# Autodesk Inventor assembly: Assembly1
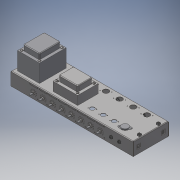
[picture p0: Inventor's stored thumbnail of the model, 180x180]
Saved by Autodesk Inventor 2016 (Build 200138000, 138)
## iProperties
Created: 2015-10-14
Part Number: Assembly1
Document SubType Name: Assembly
Designer: jeremyhale
Author: jeremyhale
## Documents named in this file (33)
- \\psf\Home\Documents\Poorhouse\git\p0001\chassis.iam
- chassis.iam
- \\psf\Home\Documents\Poorhouse\git\p0001\tube socket 8 pin.ipt
- \\psf\Home\Documents\Poorhouse\git\p0001\tube socket 9 pin.ipt
- \\psf\Home\Documents\Poorhouse\git\p0001\xmfr power.ipt
- \\psf\Home\Documents\Poorhouse\git\p0001\xmfr output.ipt
- \\psf\Home\Documents\Inventor\Content Center Files\R2016\en-US\AS 1474(1)\AS 1474 - M3(1).ipt
- \\psf\Home\Documents\Poorhouse\git\p0001\iec320_703W-00_04.ipt
- \\psf\Home\Documents\Inventor\Content Center Files\R2016\en-US\AS 1427(07)\AS 1427 - M3 x 10(6) II.ipt
- \\psf\Home\Documents\Poorhouse\git\p0001\Toggle Large A.ipt
- \\psf\Home\Documents\Poorhouse\git\p0001\AUDIO JACK 2.ipt
- \\psf\Home\Documents\Poorhouse\git\p0001\Bussman fuse holder HKP - 0,25'' X 1,25''.ipt
- \\psf\Home\Documents\Poorhouse\git\p0001\cage nut m6.iam
- \\psf\Home\Documents\Poorhouse\git\p0001\PEC11R-4220F-S0024.ipt
- \\psf\Home\Documents\Inventor\Content Center Files\R2016\en-US\UNI 5590  A\UNI 5590 - A M7.ipt
- \\psf\Home\Documents\Inventor\Content Center Files\R2016\en-US\BS 4320(2)\BS 4320 - M7 (Form B).ipt
- \\psf\Home\Documents\Poorhouse\git\p0001\rotary control.iam
- \\psf\Home\Documents\Poorhouse\git\p0001\Standoff 7mm M2 Wurth 9774070243R.ipt
- \\psf\Home\Documents\Poorhouse\git\p0001\chassis\Design Accelerator\Bolted Connection2.iam
- \\psf\Home\Documents\Poorhouse\git\p0001\chassis\Design Accelerator\Bolted Connection3.iam
- \\psf\Home\Documents\Poorhouse\git\p0001\chassis\Design Accelerator\Bolted Connection4.iam
- \\psf\Home\Documents\Poorhouse\git\p0001\chassis\Design Accelerator\Bolted Connection5.iam
- \\psf\Home\Documents\Poorhouse\git\p0001\chassis\Design Accelerator\Bolted Connection8.iam
- \\psf\Home\Documents\Poorhouse\git\p0001\chassis-weld.iam
- \\psf\Home\Documents\Poorhouse\git\p0001\octal assembly.ipt
- \\psf\Home\Documents\Poorhouse\git\p0001\chassis\Design Accelerator\Bolted Connection6.iam
- \\psf\Home\Documents\Poorhouse\git\p0001\el34 assembly_r1.ipt
- \\psf\Home\Documents\Poorhouse\git\p0001\chassis\Design Accelerator\Bolted Connection7.iam
- \\psf\Home\Documents\Poorhouse\git\p0001\chassis\Design Accelerator\Bolted Connection9.iam
- \\psf\Home\Documents\Poorhouse\git\p0001\Noval socket.ipt
- \\psf\Home\Documents\Poorhouse\git\p0001\12ax7_complete.ipt
- \\psf\Home\Documents\Poorhouse\git\p0001\chassis\Design Accelerator\Bolted Connection10.iam
- \\psf\Home\Documents\Poorhouse\git\p0001\chassis\Design Accelerator\Bolted Connection14.iam
## Components (204 placed, 25 different names)
1. xmfr power:1 — Mate:55, Mate:77, Flush:7, Flush:8, Mate:108, Mate:109
2. xmfr output:1 — Mate:76, Mate:77, Flush:6, Mate:110, Mate:111
3. Bussman fuse holder HKP - 0,25'' X 1,25'':1
4. PowerSwitch
5. chassis-weld:1 [sub-assembly] — Angle:1, Rotational:29, Rotational:30, Insert:43, Angle:2, Rigid:32, Insert:44, Angle:3, Insert:45, Angle:4, Mate:55, Mate:76, Flush:6, Flush:7, Flush:8, Mate:112, Mate:113, Mate:114, Mate:115, Mate:116, Mate:117, Mate:118, Rigid:36, Mate:119, Mate:120
6. big preamp tube socket — Insert:44, Angle:3, Mate:51, Mate:52
7. Bolted Connection:113 [sub-assembly] — Mate:108, Mate:109
8. Bolted Connection:117 [sub-assembly] — Mate:110, Mate:111
9. iec320_703W-00_04:1 — Mate:6, Mate:7
10. AS 1427 Z - Metric M3 x 10:2 — Mate:6, Mate:10
11. AS 1427 Z - Metric M3 x 10:1 — Mate:7, Mate:12
12. AS 1474 - Metric M3:5 — Mate:10
13. AS 1474 - Metric M3:6 — Mate:12
14. Input Jack
15. AUDIO JACK 2:5
16. Bolted Connection:4 [sub-assembly] — Mate:38
17. Bolted Connection:3 [sub-assembly] — Mate:30
18. Bolted Connection:2 [sub-assembly] — Mate:32
19. Bolted Connection:1 [sub-assembly] — Mate:34
20. Standoff 7mm M2 Wurth 9774070243R:4 — Insert:42, Mate:38
21. Standoff 7mm M2 Wurth 9774070243R:3 — Insert:41, Mate:32
22. Standoff 7mm M2 Wurth 9774070243R:2 — Insert:40, Mate:30
23. Standoff 7mm M2 Wurth 9774070243R:1 — Insert:39, Mate:34
24. rotary control:1 [sub-assembly] — Insert:39, Insert:40, Insert:41, Insert:42, Angle:1, Cylindrical:1, Mate:39, Mate:40
25. BS 4320 Form AB M7 (Form B):1 — Mate:15, Mate:18
26. UNI 5590 A A M7:1 — Mate:17, Mate:18
27. PEC11R-4220F-S0024:1 — Mate:15, Mate:17, Cylindrical:1
28. Bolted Connection:37 [sub-assembly]
29. Bolted Connection:38 [sub-assembly]
30. Bolted Connection:39 [sub-assembly]
31. Bolted Connection:40 [sub-assembly]
32. Standoff 7mm M2 Wurth 9774070243R:5
33. Standoff 7mm M2 Wurth 9774070243R:6
34. Standoff 7mm M2 Wurth 9774070243R:7
35. Standoff 7mm M2 Wurth 9774070243R:8
36. rotary control:2 [sub-assembly]
37. BS 4320 Form AB M7 (Form B):2
38. UNI 5590 A A M7:2
39. PEC11R-4220F-S0024:2
40. Bolted Connection:45 [sub-assembly]
41. Bolted Connection:46 [sub-assembly]
42. Bolted Connection:47 [sub-assembly]
43. Bolted Connection:48 [sub-assembly]
44. Standoff 7mm M2 Wurth 9774070243R:9
45. Standoff 7mm M2 Wurth 9774070243R:10
46. Standoff 7mm M2 Wurth 9774070243R:11
47. Standoff 7mm M2 Wurth 9774070243R:12
48. rotary control:3 [sub-assembly]
49. BS 4320 Form AB M7 (Form B):3
50. UNI 5590 A A M7:3
51. PEC11R-4220F-S0024:3
52. Bolted Connection:53 [sub-assembly]
53. Bolted Connection:54 [sub-assembly]
54. Bolted Connection:55 [sub-assembly]
55. Bolted Connection:56 [sub-assembly]
56. Standoff 7mm M2 Wurth 9774070243R:13
57. Standoff 7mm M2 Wurth 9774070243R:14
58. Standoff 7mm M2 Wurth 9774070243R:15
59. Standoff 7mm M2 Wurth 9774070243R:16
60. rotary control:4 [sub-assembly]
61. BS 4320 Form AB M7 (Form B):4
62. UNI 5590 A A M7:4
63. PEC11R-4220F-S0024:4
64. Bolted Connection:61 [sub-assembly]
65. Bolted Connection:62 [sub-assembly]
66. Bolted Connection:63 [sub-assembly]
67. Bolted Connection:64 [sub-assembly]
68. Standoff 7mm M2 Wurth 9774070243R:17
69. Standoff 7mm M2 Wurth 9774070243R:18
70. Standoff 7mm M2 Wurth 9774070243R:19
71. Standoff 7mm M2 Wurth 9774070243R:20
72. rotary control:5 [sub-assembly]
73. BS 4320 Form AB M7 (Form B):5
74. UNI 5590 A A M7:5
75. PEC11R-4220F-S0024:5
76. Bolted Connection:69 [sub-assembly]
77. Bolted Connection:70 [sub-assembly]
78. Bolted Connection:71 [sub-assembly]
79. Bolted Connection:72 [sub-assembly]
80. Standoff 7mm M2 Wurth 9774070243R:21
81. Standoff 7mm M2 Wurth 9774070243R:22
82. Standoff 7mm M2 Wurth 9774070243R:23
83. Standoff 7mm M2 Wurth 9774070243R:24
84. rotary control:6 [sub-assembly]
85. BS 4320 Form AB M7 (Form B):6
86. UNI 5590 A A M7:6
87. PEC11R-4220F-S0024:6
88. Bolted Connection:77 [sub-assembly]
89. Bolted Connection:78 [sub-assembly]
90. Bolted Connection:79 [sub-assembly]
91. Bolted Connection:80 [sub-assembly]
92. Standoff 7mm M2 Wurth 9774070243R:25
93. Standoff 7mm M2 Wurth 9774070243R:26
94. Standoff 7mm M2 Wurth 9774070243R:27
95. Standoff 7mm M2 Wurth 9774070243R:28
96. rotary control:7 [sub-assembly]
97. BS 4320 Form AB M7 (Form B):7
98. UNI 5590 A A M7:7
99. PEC11R-4220F-S0024:7
100. Bolted Connection:85 [sub-assembly]
101. Bolted Connection:86 [sub-assembly]
102. Bolted Connection:87 [sub-assembly]
103. Bolted Connection:88 [sub-assembly]
104. Standoff 7mm M2 Wurth 9774070243R:29
105. Standoff 7mm M2 Wurth 9774070243R:30
106. Standoff 7mm M2 Wurth 9774070243R:31
107. Standoff 7mm M2 Wurth 9774070243R:32
108. rotary control:8 [sub-assembly]
109. BS 4320 Form AB M7 (Form B):8
110. UNI 5590 A A M7:8
111. PEC11R-4220F-S0024:8
112. AUDIO JACK 2:6 — Rotational:29
113. AUDIO JACK 2:7
114. AUDIO JACK 2:8
115. jack speaker — Rotational:30
116. AUDIO JACK 2:9
117. AUDIO JACK 2:10
118. tube socket 8 pin:1 — Insert:43, Angle:2, Mate:53, Mate:54
119. octal assembly:1 — Rigid:32, Rigid:33
120. el34 assembly_r1:1 — Rigid:33
121. tube socket 8 pin:8
122. octal assembly:2
123. el34 assembly_r1:2
124. tube socket 8 pin:9
125. octal assembly:3
126. el34 assembly_r1:3
127. tube socket 8 pin:10
128. octal assembly:4
129. el34 assembly_r1:4
130. tube socket 8 pin:11
131. octal assembly:5
132. el34 assembly_r1:5
133. tube socket 8 pin:12
134. octal assembly:6
135. el34 assembly_r1:6
136. Bolted Connection:105 [sub-assembly] — Mate:51, Mate:52
137. Bolted Connection:106 [sub-assembly]
138. tube socket 9 pin:1 — Insert:45, Angle:4, Mate:49, Mate:50
139. Noval socket:1 — Rigid:35, Rigid:36
140. 12ax7_complete:1 — Rigid:35
141. tube socket 9 pin:2
142. Noval socket:2
143. 12ax7_complete:2
144. tube socket 9 pin:3
145. Noval socket:3
146. 12ax7_complete:3
147. cage nut m6:5 [sub-assembly] — Mate:112, Mate:113, Mate:114
148. cage nut m6:9 [sub-assembly]
149. cage nut m6:7 [sub-assembly] — Mate:115, Mate:116, Mate:117
150. cage nut m6:10 [sub-assembly]
151. cage nut m6:1 [sub-assembly] — Mate:118, Mate:119, Mate:120
152. cage nut m6:11 [sub-assembly]
153. cage nut m6:12 [sub-assembly]
154. cage nut m6:13 [sub-assembly]
155. Bolted Connection:33 [sub-assembly] — Mate:39, Mate:40
156. Bolted Connection:34 [sub-assembly]
157. Bolted Connection:35 [sub-assembly]
158. Bolted Connection:36 [sub-assembly]
159. Bolted Connection:41 [sub-assembly]
160. Bolted Connection:42 [sub-assembly]
161. Bolted Connection:43 [sub-assembly]
162. Bolted Connection:44 [sub-assembly]
163. Bolted Connection:49 [sub-assembly]
164. Bolted Connection:50 [sub-assembly]
165. Bolted Connection:51 [sub-assembly]
166. Bolted Connection:52 [sub-assembly]
167. Bolted Connection:57 [sub-assembly]
168. Bolted Connection:58 [sub-assembly]
169. Bolted Connection:59 [sub-assembly]
170. Bolted Connection:60 [sub-assembly]
171. Bolted Connection:65 [sub-assembly]
172. Bolted Connection:66 [sub-assembly]
173. Bolted Connection:67 [sub-assembly]
174. Bolted Connection:68 [sub-assembly]
175. Bolted Connection:73 [sub-assembly]
176. Bolted Connection:74 [sub-assembly]
177. Bolted Connection:75 [sub-assembly]
178. Bolted Connection:76 [sub-assembly]
179. Bolted Connection:81 [sub-assembly]
180. Bolted Connection:82 [sub-assembly]
181. Bolted Connection:83 [sub-assembly]
182. Bolted Connection:84 [sub-assembly]
183. Bolted Connection:89 [sub-assembly]
184. Bolted Connection:90 [sub-assembly]
185. Bolted Connection:91 [sub-assembly]
186. Bolted Connection:92 [sub-assembly]
187. Bolted Connection:93 [sub-assembly] — Mate:53, Mate:54
188. Bolted Connection:94 [sub-assembly]
189. Bolted Connection:95 [sub-assembly]
190. Bolted Connection:96 [sub-assembly]
191. Bolted Connection:97 [sub-assembly]
192. Bolted Connection:98 [sub-assembly]
193. Bolted Connection:99 [sub-assembly]
194. Bolted Connection:100 [sub-assembly]
195. Bolted Connection:101 [sub-assembly]
196. Bolted Connection:102 [sub-assembly]
197. Bolted Connection:103 [sub-assembly]
198. Bolted Connection:104 [sub-assembly]
199. Bolted Connection:107 [sub-assembly] — Mate:49, Mate:50
200. Bolted Connection:108 [sub-assembly]
201. Bolted Connection:109 [sub-assembly]
202. Bolted Connection:110 [sub-assembly]
203. Bolted Connection:111 [sub-assembly]
204. Bolted Connection:112 [sub-assembly]
## Component patterns: jacks input (2 elements), controls (8 elements), jacks fx (3 elements), jacks speaker (3 elements), big tubes (6 elements), big preamp tube screws (2 elements), small preamp tubes (3 elements), (2 elements, first: cage nut m6:5), (2 elements, first: cage nut m6:7), (4 elements, first: cage nut m6:1), (4 elements, first: Bolted Connection:33), Component Pattern 21:2 (4 elements), Component Pattern 21:3 (4 elements), Component Pattern 21:4 (4 elements), Component Pattern 21:5 (4 elements), Component Pattern 21:6 (4 elements), Component Pattern 21:7 (4 elements), Component Pattern 21:8 (4 elements), big tube socket screws (2 elements), big tube socket screws:2 (2 elements), big tube socket screws:3 (2 elements), big tube socket screws:4 (2 elements), big tube socket screws:5 (2 elements), big tube socket screws:6 (2 elements), small tube screws (2 elements), small tube screws:2 (2 elements), small tube screws:3 (2 elements)
## Relationships (74: Mate 44, Insert 7, RevoluteJoint 6, WeldJoint 6, Flush 6, Angle 4, CylindricalJoint 1)
- [RevoluteJoint]: chassis-weld:1 ↔ iec320_703W-00_04:1
- [RevoluteJoint]: chassis-weld:1 ↔ iec320_703W-00_04:1
- Mate:6: iec320_703W-00_04:1 ↔ AS 1427 Z - Metric M3 x 10:2
- Mate:7: iec320_703W-00_04:1 ↔ AS 1427 Z - Metric M3 x 10:1
- Mate:10: AS 1427 Z - Metric M3 x 10:2 ↔ AS 1474 - Metric M3:5
- [Mate]: chassis-weld:1 ↔ AS 1474 - Metric M3:5
- Mate:12: AS 1427 Z - Metric M3 x 10:1 ↔ AS 1474 - Metric M3:6
- [Mate]: chassis-weld:1 ↔ AS 1474 - Metric M3:6
- [WeldJoint]: Bussman fuse holder HKP - 0,25'' X 1,25'':1 ↔ chassis-weld:1
- [WeldJoint]: PowerSwitch ↔ chassis-weld:1
- [Flush]: chassis-weld:1
- [Flush]: chassis-weld:1
- [Flush]: chassis-weld:1
- Mate:15: BS 4320 Form AB M7 (Form B):1 ↔ PEC11R-4220F-S0024:1
- [Mate]: chassis-weld:1 ↔ BS 4320 Form AB M7 (Form B):1
- Mate:17: UNI 5590 A A M7:1 ↔ PEC11R-4220F-S0024:1
- Mate:18: BS 4320 Form AB M7 (Form B):1 ↔ UNI 5590 A A M7:1
- Insert:39: Standoff 7mm M2 Wurth 9774070243R:1 ↔ rotary control:1
- Insert:40: Standoff 7mm M2 Wurth 9774070243R:2 ↔ rotary control:1
- Insert:41: Standoff 7mm M2 Wurth 9774070243R:3 ↔ rotary control:1
- Insert:42: Standoff 7mm M2 Wurth 9774070243R:4 ↔ rotary control:1
- [Mate]: chassis-weld:1 ↔ Standoff 7mm M2 Wurth 9774070243R:1
- [Mate]: chassis-weld:1 ↔ Standoff 7mm M2 Wurth 9774070243R:4
- Angle:1 (0 deg): chassis-weld:1 ↔ rotary control:1
- Cylindrical:1: rotary control:1 ↔ PEC11R-4220F-S0024:1
- [Mate]: chassis-weld:1 ↔ Bolted Connection:3
- Mate:30: Bolted Connection:3 ↔ Standoff 7mm M2 Wurth 9774070243R:2
- [Mate]: chassis-weld:1 ↔ Bolted Connection:2
- Mate:32: Bolted Connection:2 ↔ Standoff 7mm M2 Wurth 9774070243R:3
- [Mate]: chassis-weld:1 ↔ Bolted Connection:1
- Mate:34: Bolted Connection:1 ↔ Standoff 7mm M2 Wurth 9774070243R:1
- [RevoluteJoint]: chassis-weld:1 ↔ Input Jack
- [RevoluteJoint]: chassis-weld:1 ↔ PEC11R-4220F-S0024:1
- [Mate]: chassis-weld:1 ↔ Bolted Connection:4
- Mate:38: Bolted Connection:4 ↔ Standoff 7mm M2 Wurth 9774070243R:4
- Mate:39: rotary control:1 ↔ Bolted Connection:33
- Mate:40: rotary control:1 ↔ Bolted Connection:33
- Rotational:29 [RevoluteJoint]: chassis-weld:1 ↔ AUDIO JACK 2:6
- Rotational:30 [RevoluteJoint]: chassis-weld:1 ↔ jack speaker
- Insert:43: chassis-weld:1 ↔ tube socket 8 pin:1
- Angle:2 (120 deg): chassis-weld:1 ↔ tube socket 8 pin:1
- Rigid:32 [WeldJoint]: chassis-weld:1 ↔ octal assembly:1
- Rigid:33 [WeldJoint]: octal assembly:1 ↔ el34 assembly_r1:1
- Insert:44: chassis-weld:1 ↔ big preamp tube socket
- Angle:3 (30 deg): chassis-weld:1 ↔ big preamp tube socket
- Insert:45: chassis-weld:1 ↔ tube socket 9 pin:1
- Angle:4 (30 deg): chassis-weld:1 ↔ tube socket 9 pin:1
- Mate:49: tube socket 9 pin:1 ↔ Bolted Connection:107
- Mate:50: tube socket 9 pin:1 ↔ Bolted Connection:107
- Mate:51: big preamp tube socket ↔ Bolted Connection:105
- Mate:52: big preamp tube socket ↔ Bolted Connection:105
- Mate:53: tube socket 8 pin:1 ↔ Bolted Connection:93
- Mate:54: tube socket 8 pin:1 ↔ Bolted Connection:93
- Rigid:35 [WeldJoint]: Noval socket:1 ↔ 12ax7_complete:1
- Mate:55 (3.175 mm): xmfr power:1 ↔ chassis-weld:1
- Mate:76 (3.175 mm): xmfr output:1 ↔ chassis-weld:1
- Mate:77 (63.5 mm): xmfr power:1 ↔ xmfr output:1
- Flush:6 (12.7 mm): xmfr output:1 ↔ chassis-weld:1
- Flush:7 (19.05 mm): xmfr power:1 ↔ chassis-weld:1
- Flush:8 (12.7 mm): xmfr power:1 ↔ chassis-weld:1
- Mate:108: xmfr power:1 ↔ Bolted Connection:113
- Mate:109: xmfr power:1 ↔ Bolted Connection:113
- Mate:110: xmfr output:1 ↔ Bolted Connection:117
- Mate:111: xmfr output:1 ↔ Bolted Connection:117
- Mate:112 (0.508 mm): chassis-weld:1 ↔ cage nut m6:5
- Mate:113 (1.27 mm): chassis-weld:1 ↔ cage nut m6:5
- Mate:114: chassis-weld:1 ↔ cage nut m6:5
- Mate:115: chassis-weld:1 ↔ cage nut m6:7
- Mate:116 (0.508 mm): chassis-weld:1 ↔ cage nut m6:7
- Mate:117 (1.27 mm): chassis-weld:1 ↔ cage nut m6:7
- Mate:118: chassis-weld:1 ↔ cage nut m6:1
- Rigid:36 [WeldJoint]: chassis-weld:1 ↔ Noval socket:1
- Mate:119 (0.508 mm): chassis-weld:1 ↔ cage nut m6:1
- Mate:120 (1.27 mm): chassis-weld:1 ↔ cage nut m6:1
## Named parameters: tubeAngle = 30 deg, xfmrPowerOffsetZ = 3.175 mm, xmfrOutputOffsetZ = 3.175 mm, xmfrOutputOffsetFromPwr = 63.5 mm, xfmrOutputOffsetFromChassis = 12.7 mm, xmfrPowerOffsetX = 19.05 mm, xfmrPowerOffsetY = 12.7 mm
